# Autodesk Inventor assembly: ServoShaftCouplerAssembly
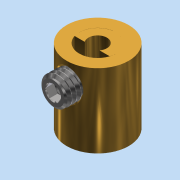
[picture p0: Inventor's stored thumbnail of the model, 180x180]
Saved by Autodesk Inventor 2017 (Build 210142000, 142)
## iProperties
Created: 2017-11-01
Part Number: ServoShaftCouplerAssembly
Document SubType Name: Assembly
Designer: Derek Wider
Author: Derek Wider
## Documents named in this file (4)
- E:\OneDrive\Documents\Other Projects\Submarine\CAD\midships\AftServoSection\ServoShaftCoupler\ServoShaftCouplerAssembly.iam
- E:\OneDrive\Documents\Other Projects\Submarine\CAD\midships\AftServoSection\ServoShaftCoupler\ShaftCoupler.ipt
- E:\OneDrive\Documents\Other Projects\Submarine\CAD\midships\AftServoSection\ServoShaftCoupler\ShaftCollar.ipt
- E:\OneDrive\Documents\Other Projects\Submarine\CAD\midships\AftServoSection\ServoShaftCoupler\SetScrewLong.ipt
## Components (3 placed, 3 different names)
1. ShaftCoupler:1 — Mate:2, Mate:3, Mate:4, Angle:1
2. ShaftCollar:1 — Mate:2, Mate:3, Flush:1
3. SetScrewLong:1 — Mate:4, Flush:1, Angle:1
## Relationships (5: Mate 3, Flush 1, Angle 1)
- Mate:2: ShaftCoupler:1 ↔ ShaftCollar:1
- Mate:3: ShaftCoupler:1 ↔ ShaftCollar:1
- Mate:4: ShaftCoupler:1 ↔ SetScrewLong:1
- Flush:1 (-6.731 mm): ShaftCollar:1 ↔ SetScrewLong:1
- Angle:1 (0 deg): ShaftCoupler:1 ↔ SetScrewLong:1
